# Autodesk Inventor assembly: waveshare-10-version
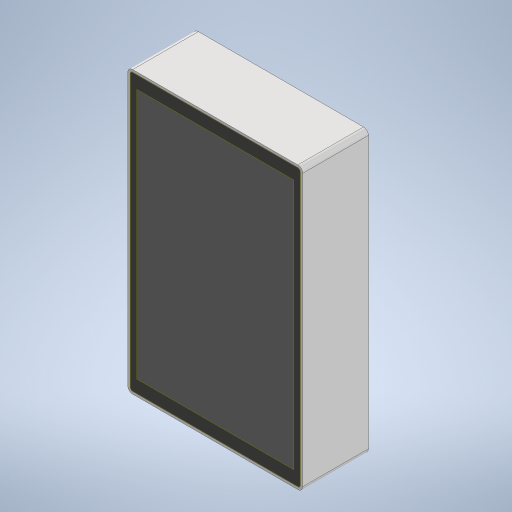
[picture p0: Inventor's stored thumbnail of the model, 512x512]
Saved by Autodesk Inventor 2024 (Build 280153000, 153)
## iProperties
Created: 2024-11-18
Part Number: waveshare-10-version
Document SubType Name: Assembly
Designer: Stefano
Author: Stefano
## Documents named in this file (5)
- C:\Users\Stefano\Documents\Inventor\Provvedo\inventor-dro-case\waveshare-10-version\waveshare-10-version.iam
- C:\Users\Stefano\Documents\Inventor\Provvedo\inventor-dro-case\waveshare-10-version\10_1inch-dsi-lcd_c_New\10_1inch-dsi-lcd_c_New.ipt
- C:\Users\Stefano\Documents\Inventor\Provvedo\inventor-dro-case\waveshare-10-version\enclosure-body.ipt
- C:\Users\Stefano\Documents\Inventor\Provvedo\inventor-dro-case\waveshare-10-version\Raspberry Pi 3 .ipt
- C:\Users\Stefano\Documents\Inventor\Provvedo\inventor-dro-case\waveshare-10-version\Rotary Controller V1.ipt
## Components (4 placed, 4 different names)
1. 10_1inch-dsi-lcd_c_New:1 — Flush:1, Flush:2, Flush:3, Flush:5, Cylindrical:1, Mate:2
2. enclosure-body:1 — Flush:1, Flush:2, Flush:4, Mate:3, Mate:4
3. Raspberry Pi 3 :1 — Mate:1, Cylindrical:1, Mate:2
4. Rotary Controller V1:1 — Mate:3, Mate:4
## Relationships (10: Flush 5, Mate 4, CylindricalJoint 1)
- Flush:1: 10_1inch-dsi-lcd_c_New:1 ↔ enclosure-body:1
- Flush:2: 10_1inch-dsi-lcd_c_New:1 ↔ enclosure-body:1
- Flush:3 (1 mm): 10_1inch-dsi-lcd_c_New:1
- Flush:4: enclosure-body:1
- Flush:5 (8 mm): 10_1inch-dsi-lcd_c_New:1
- Mate:1: Raspberry Pi 3 :1
- Cylindrical:1: 10_1inch-dsi-lcd_c_New:1 ↔ Raspberry Pi 3 :1
- Mate:2: 10_1inch-dsi-lcd_c_New:1 ↔ Raspberry Pi 3 :1
- Mate:3: enclosure-body:1 ↔ Rotary Controller V1:1
- Mate:4 (6.35 mm): enclosure-body:1 ↔ Rotary Controller V1:1
